# Autodesk Inventor assembly: GarageAndBracketFlatBracket
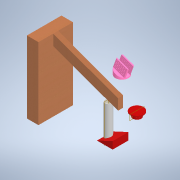
[picture p0: Inventor's stored thumbnail of the model, 180x180]
Saved by Autodesk Inventor 2022.2 (Build 262287000, 287)
## iProperties
Created: 2021-11-26
Part Number: GarageAndBracketFlatBracket
Document SubType Name: Assembly
Designer: robst
Author: robst
## Documents named in this file (6)
- C:\git\CAD-Development\robSteele\ShapeWays\GlobalMeteorNetwork\GarageAndBracketFlatBracket.iam
- C:\git\CAD-Development\robSteele\ShapeWays\GlobalMeteorNetwork\GarageSegment.ipt
- C:\git\CAD-Development\robSteele\ShapeWays\GlobalMeteorNetwork\pvcBracketUpperPortionV02.ipt
- C:\git\CAD-Development\robSteele\ShapeWays\GlobalMeteorNetwork\2inchPvcForBracket.ipt
- C:\git\CAD-Development\robSteele\ShapeWays\GlobalMeteorNetwork\topAttachementFor2InchPvcPipe.ipt
- C:\git\CAD-Development\robSteele\ShapeWays\GlobalMeteorNetwork\bottomAttachementFor2InchPvcPipe.ipt
## Components (5 placed, 5 different names)
1. GarageSegment:1 — Mate:13, Mate:14
2. pvcBracketUpperPortionV02:1 — Mate:13, Mate:14
3. 2inchPvcForBracket:1 — Insert:1
4. topAttachementFor2InchPvcPipe:1
5. bottomAttachementFor2InchPvcPipe:1 — Insert:1
## Relationships (3: Mate 2, Insert 1)
- Mate:13: GarageSegment:1 ↔ pvcBracketUpperPortionV02:1
- Mate:14: GarageSegment:1 ↔ pvcBracketUpperPortionV02:1
- Insert:1: 2inchPvcForBracket:1 ↔ bottomAttachementFor2InchPvcPipe:1
